# Autodesk Inventor assembly: вт
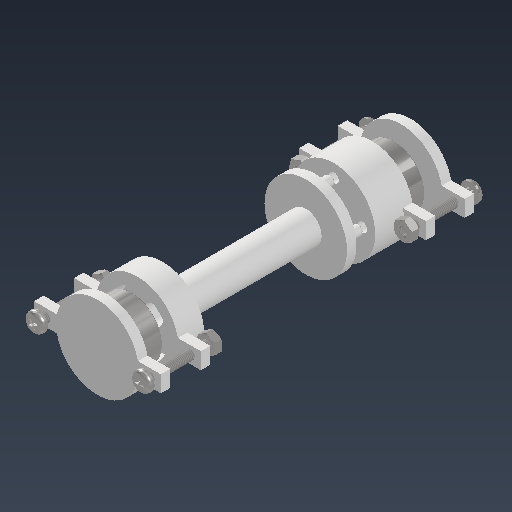
[picture p0: Inventor's stored thumbnail of the model, 512x512]
Saved by Autodesk Inventor 2025 (Build 290162000, 162)
## iProperties
Created: 2025-03-14
Part Number: вт
Document SubType Name: Assembly
Designer: GameHD
Author: GameHD
## Documents named in this file (7)
- C:\Users\GameHD\Desktop\Phantom 16950\вт.iam
- C:\Users\GameHD\Desktop\Phantom 16950\вт3.ipt
- C:\Users\GameHD\Desktop\Phantom 16950\вт1.ipt
- C:\Users\GameHD\Desktop\Phantom 16950\вт2.ipt
- C:\Users\GameHD\Desktop\Phantom 16950\BS 290 SKF - SKF 626-RZ.ipt
- C:\Users\GameHD\Documents\Inventor\Content Center Files\R2025\ru-RU\AS 1427(05)\AS 1427 - M3 x 20(5) II.ipt
- C:\Users\GameHD\Documents\Inventor\Content Center Files\R2025\ru-RU\BS 3692(1)\BS 3692 - M3(1).ipt
## Components (14 placed, 6 different names)
1. вт3:1 — Совмещение:5, Совмещение:6, Совмещение:9, Совмещение:10
2. вт1:1 — Совмещение:1, Совмещение:2, Совмещение:5, Совмещение:6, Совмещение:7
3. вт2:1 — Совмещение:1, Совмещение:2, Совмещение:3, Совмещение:4, Совмещение:8
4. вт3:2 — Совмещение:3, Совмещение:4, Совмещение:11, Совмещение:12
5. BS 290 SKF - SKF 626-RZ:1 — Совмещение:7
6. BS 290 SKF - SKF 626-RZ:2 — Совмещение:8
7. AS 1427 H - метрическая M3 x 20:1 — Совмещение:9, Совмещение:13
8. AS 1427 H - метрическая M3 x 20:2 — Совмещение:10, Совмещение:14
9. AS 1427 H - метрическая M3 x 20:3 — Совмещение:11, Совмещение:16
10. AS 1427 H - метрическая M3 x 20:4 — Совмещение:12, Совмещение:15
11. BS 3692 - метрическая M3:1 — Совмещение:14
12. BS 3692 - метрическая M3:2 — Совмещение:13
13. BS 3692 - метрическая M3:3 — Совмещение:16
14. BS 3692 - метрическая M3:4 — Совмещение:15
## Relationships (16: Mate 16)
- Совмещение:1 [Mate]: вт1:1 ↔ вт2:1
- Совмещение:2 [Mate]: вт1:1 ↔ вт2:1
- Совмещение:3 [Mate]: вт2:1 ↔ вт3:2
- Совмещение:4 [Mate]: вт2:1 ↔ вт3:2
- Совмещение:5 [Mate]: вт3:1 ↔ вт1:1
- Совмещение:6 [Mate]: вт3:1 ↔ вт1:1
- Совмещение:7 [Mate]: вт1:1 ↔ BS 290 SKF - SKF 626-RZ:1
- Совмещение:8 [Mate]: вт2:1 ↔ BS 290 SKF - SKF 626-RZ:2
- Совмещение:9 [Mate]: вт3:1 ↔ AS 1427 H - метрическая M3 x 20:1
- Совмещение:10 [Mate]: вт3:1 ↔ AS 1427 H - метрическая M3 x 20:2
- Совмещение:11 [Mate]: вт3:2 ↔ AS 1427 H - метрическая M3 x 20:3
- Совмещение:12 [Mate]: вт3:2 ↔ AS 1427 H - метрическая M3 x 20:4
- Совмещение:13 [Mate]: AS 1427 H - метрическая M3 x 20:1 ↔ BS 3692 - метрическая M3:2
- Совмещение:14 [Mate]: AS 1427 H - метрическая M3 x 20:2 ↔ BS 3692 - метрическая M3:1
- Совмещение:15 [Mate]: AS 1427 H - метрическая M3 x 20:4 ↔ BS 3692 - метрическая M3:4
- Совмещение:16 [Mate]: AS 1427 H - метрическая M3 x 20:3 ↔ BS 3692 - метрическая M3:3
